# Autodesk Inventor assembly: Assembly1
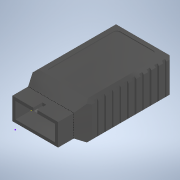
[picture p0: Inventor's stored thumbnail of the model, 180x180]
Saved by Autodesk Inventor 2021 (Build 250183000, 183)
## iProperties
Created: 2020-12-01
Part Number: Assembly1
Document SubType Name: Assembly
Designer: Blake
Author: Blake
## Documents named in this file (3)
- F:\Users\Blake\Documents\Inventor\ODB2\Assembly1.iam
- F:\Users\Blake\Documents\Inventor\ODB2\Main_Housing_Base.ipt
- F:\Users\Blake\Documents\Inventor\ODB2\Main_Housing_Cap.ipt
## Components (2 placed, 2 different names)
1. Main_Housing_Base:1 — Flush:1, Mate:1, Mate:2
2. Main_Housing_Cap:1 — Flush:1, Mate:1, Mate:2
## Relationships (3: Mate 2, Flush 1)
- Flush:1: Main_Housing_Base:1 ↔ Main_Housing_Cap:1
- Mate:1 (0.381 mm): Main_Housing_Base:1 ↔ Main_Housing_Cap:1
- Mate:2 (0.381 mm): Main_Housing_Base:1 ↔ Main_Housing_Cap:1
